# Autodesk Inventor assembly: ENSAMBLE_2
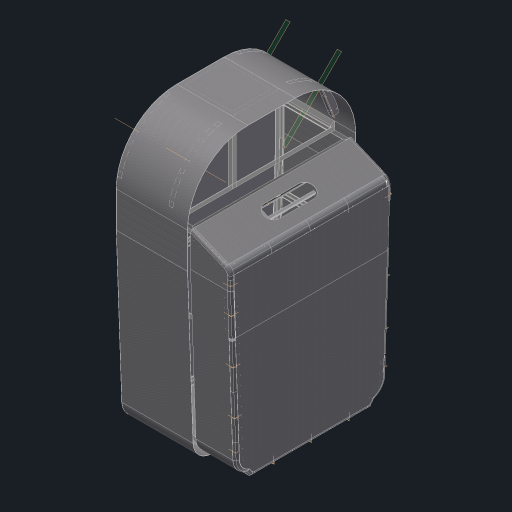
[picture p0: Inventor's stored thumbnail of the model, 512x512]
Saved by Autodesk Inventor 2024.3 (Build 283343000, 343)
## iProperties
Created: 2024-06-14
Part Number: ENSAMBLE_2
Material: Generic
Document SubType Name: Assembly
Designer: Niler
Author: Niler
## Documents named in this file (21)
- C:\Users\Niler\OneDrive\Escritorio\RECICLADOR\RECICLADOR_MODELO_3D\VERSION_3_COMPLETA\ENSAMBLE_2.iam
- C:\Users\Niler\OneDrive\Escritorio\RECICLADOR\RECICLADOR_MODELO_3D\VERSION_3_COMPLETA\CARCASA_ESTRUCTURA_Y_CHAPAS_2.iam
- C:\Users\Niler\OneDrive\Escritorio\RECICLADOR\RECICLADOR_MODELO_3D\VERSION_3_COMPLETA\PIEZAS_CHAPAS_ALUMINIO\CARCASA_ALUM_1.ipt
- C:\Users\Niler\OneDrive\Escritorio\RECICLADOR\RECICLADOR_MODELO_3D\VERSION_3_COMPLETA\ESQUINAS\ESQUINA_REDONDEADA_R20_P10.ipt
- C:\Users\Niler\OneDrive\Escritorio\RECICLADOR\RECICLADOR_MODELO_3D\VERSION_3_COMPLETA\ESQUINAS\ESQUINA_REDONDEADA_R20_P11.ipt
- C:\Users\Niler\OneDrive\Escritorio\RECICLADOR\RECICLADOR_MODELO_3D\VERSION_3_COMPLETA\ESQUINAS\ESQUINA_REDONDEADA_R20_P12.ipt
- C:\Users\Niler\OneDrive\Escritorio\RECICLADOR\RECICLADOR_MODELO_3D\VERSION_3_COMPLETA\NUEVAS_CHAPAS_ALUMINIO\CHAPA_1.ipt
- C:\Users\Niler\OneDrive\Escritorio\RECICLADOR\RECICLADOR_MODELO_3D\VERSION_3_COMPLETA\NUEVAS_CHAPAS_ALUMINIO\CHAPA_2.ipt
- C:\Users\Niler\OneDrive\Escritorio\RECICLADOR\RECICLADOR_MODELO_3D\VERSION_3_COMPLETA\NUEVAS_CHAPAS_ALUMINIO\CHAPA_3.ipt
- C:\Users\Niler\OneDrive\Escritorio\RECICLADOR\RECICLADOR_MODELO_3D\VERSION_3_COMPLETA\ESQUINAS\ESQUINA_REDONDEADA_R20_P5.ipt
- C:\Users\Niler\OneDrive\Escritorio\RECICLADOR\RECICLADOR_MODELO_3D\VERSION_3_COMPLETA\ESQUINAS\ESQUINA_REDONDEADA_R20_P13.ipt
- C:\Users\Niler\OneDrive\Escritorio\RECICLADOR\RECICLADOR_MODELO_3D\MECANISMO DE COMPACTADO\ENSAMBLE MECANISMO DE INGRESO.iam
- C:\Users\Niler\OneDrive\Escritorio\RECICLADOR\RECICLADOR_MODELO_3D\VERSION_3_COMPLETA\CURVA_SUPERIOR_IMPR.ipt
- C:\Users\Niler\OneDrive\Escritorio\RECICLADOR\RECICLADOR_MODELO_3D\VERSION_3_COMPLETA\ESQUINAS\ESQUINA_REDONDEADA_TRASERA.ipt
- C:\Users\Niler\OneDrive\Escritorio\RECICLADOR\RECICLADOR_MODELO_3D\VERSION_3_COMPLETA\ESQUINAS\ESQUINA_REDONDEADA_TRASERA_MIR.ipt
- C:\Users\Niler\OneDrive\Escritorio\RECICLADOR\RECICLADOR_MODELO_3D\VERSION_3_COMPLETA\CURVA_SUPERIOR_IMPR_MIR.ipt
- C:\Users\Niler\OneDrive\Escritorio\RECICLADOR\RECICLADOR_MODELO_3D\VERSION_3_COMPLETA\NUEVAS_CHAPAS_ALUMINIO\CHAPA_4_v2.ipt
- C:\Users\Niler\OneDrive\Escritorio\RECICLADOR\RECICLADOR_MODELO_3D\VERSION_3_COMPLETA\NUEVAS_CHAPAS_ALUMINIO\CHAPA_4_v2_MIR.ipt
- C:\Users\Niler\OneDrive\Escritorio\RECICLADOR\RECICLADOR_MODELO_3D\VERSION_3_COMPLETA\NUEVAS_CHAPAS_ALUMINIO\CHAPA_5.ipt
- C:\Users\Niler\OneDrive\Escritorio\RECICLADOR\RECICLADOR_MODELO_3D\VERSION_3_COMPLETA\ESQUINAS\ESQUINA_REDONDEADA_R20_P12_MIR.ipt
- C:\Users\Niler\OneDrive\Escritorio\RECICLADOR\RECICLADOR_MODELO_3D\VERSION_3_COMPLETA\NUEVAS_CHAPAS_ALUMINIO\CHAPA_6.ipt
## Components (30 placed, 20 different names)
1. CARCASA_ESTRUCTURA_Y_CHAPAS_2:1 [sub-assembly] — Flush:1, Mate:2, Mate:3, Mate:6, Mate:13, Mate:14, Mate:15, Mate:17, Mate:21, Mate:22, Mate:23, Mate:30, Mate:31, Mate:32, Mate:33, Mate:34, Mate:35, Mate:38, Mate:39, Flush:12, Mate:40, Flush:16, Mate:45, Flush:17, Mate:46, Mate:50, Mate:51, Flush:18
2. CARCASA_ALUM_1:1 — Flush:1, Mate:40, Mate:41, Mate:53
3. ESQUINA_REDONDEADA_R20_P10:1 — Mate:2, Mate:4, Mate:5, Mate:6, Mate:9, Flush:2, Mate:16
4. ESQUINA_REDONDEADA_R20_P11:1 — Mate:3, Mate:4, Mate:5, Mate:36
5. ESQUINA_REDONDEADA_R20_P10:2 — Mate:9, Flush:2, Flush:5, Mate:12, Flush:11
6. ESQUINA_REDONDEADA_R20_P11:2 — Flush:11, Mate:36, Mate:37
7. ESQUINA_REDONDEADA_R20_P10:3 — Flush:5, Mate:12
8. ESQUINA_REDONDEADA_R20_P11:3 — Mate:37
9. ESQUINA_REDONDEADA_R20_P12:1 — Mate:13, Mate:14, Mate:15
10. CHAPA_1:1 — Mate:33, Mate:34, Mate:35
11. CHAPA_2:1 — Mate:18, Flush:6
12. CHAPA_3:1 — Mate:16, Mate:17, Mate:18, Flush:6
13. ESQUINA_REDONDEADA_R20_P5:1 — Mate:22, Mate:27
14. ESQUINA_REDONDEADA_R20_P5:2 — Mate:21, Mate:23, Mate:26, Flush:9
15. ESQUINA_REDONDEADA_R20_P5:3 — Mate:27
16. ESQUINA_REDONDEADA_R20_P5:4 — Mate:26, Flush:9
17. ESQUINA_REDONDEADA_R20_P13:1 — Mate:28, Flush:10, Mate:29, Mate:30
18. ESQUINA_REDONDEADA_R20_P13:2 — Mate:28, Flush:10, Mate:29, Mate:31, Mate:32
19. ENSAMBLE MECANISMO DE INGRESO:1 [sub-assembly] — Mate:38, Mate:39
20. CURVA_SUPERIOR_IMPR:1 — Flush:12, Mate:41, Mate:44, Mate:47
21. CURVA_SUPERIOR_IMPR:3 — Mate:44, Flush:16, Mate:47, Flush:19
22. ESQUINA_REDONDEADA_TRASERA:1 — Mate:45, Flush:17, Mate:46, Mate:52
23. ESQUINA_REDONDEADA_TRASERA_MIR:1
24. CURVA_SUPERIOR_IMPR_MIR:1 — Mate:48, Mate:49
25. CURVA_SUPERIOR_IMPR_MIR:2 — Mate:48, Mate:49
26. CHAPA_4_v2:1 — Mate:50, Mate:51
27. CHAPA_4_v2_MIR:1
28. CHAPA_5:1 — Mate:52, Flush:18, Mate:53
29. ESQUINA_REDONDEADA_R20_P12_MIR:1
30. CHAPA_6:1 — Flush:19
## Relationships (64: Mate 50, Flush 14)
- Flush:1: CARCASA_ESTRUCTURA_Y_CHAPAS_2:1 ↔ CARCASA_ALUM_1:1
- Mate:2: CARCASA_ESTRUCTURA_Y_CHAPAS_2:1 ↔ ESQUINA_REDONDEADA_R20_P10:1
- Mate:3: CARCASA_ESTRUCTURA_Y_CHAPAS_2:1 ↔ ESQUINA_REDONDEADA_R20_P11:1
- Mate:4: ESQUINA_REDONDEADA_R20_P10:1 ↔ ESQUINA_REDONDEADA_R20_P11:1
- Mate:5: ESQUINA_REDONDEADA_R20_P10:1 ↔ ESQUINA_REDONDEADA_R20_P11:1
- Mate:6: CARCASA_ESTRUCTURA_Y_CHAPAS_2:1 ↔ ESQUINA_REDONDEADA_R20_P10:1
- [Mate]: ESQUINA_REDONDEADA_R20_P10:2 ↔ ESQUINA_REDONDEADA_R20_P11:2
- [Mate]: ESQUINA_REDONDEADA_R20_P10:2 ↔ ESQUINA_REDONDEADA_R20_P11:2
- Mate:9: ESQUINA_REDONDEADA_R20_P10:1 ↔ ESQUINA_REDONDEADA_R20_P10:2
- Flush:2: ESQUINA_REDONDEADA_R20_P10:1 ↔ ESQUINA_REDONDEADA_R20_P10:2
- [Mate]: ESQUINA_REDONDEADA_R20_P10:3 ↔ ESQUINA_REDONDEADA_R20_P11:3
- [Mate]: ESQUINA_REDONDEADA_R20_P10:3 ↔ ESQUINA_REDONDEADA_R20_P11:3
- Flush:5: ESQUINA_REDONDEADA_R20_P10:2 ↔ ESQUINA_REDONDEADA_R20_P10:3
- Mate:12: ESQUINA_REDONDEADA_R20_P10:2 ↔ ESQUINA_REDONDEADA_R20_P10:3
- Mate:13: CARCASA_ESTRUCTURA_Y_CHAPAS_2:1 ↔ ESQUINA_REDONDEADA_R20_P12:1
- Mate:14: CARCASA_ESTRUCTURA_Y_CHAPAS_2:1 ↔ ESQUINA_REDONDEADA_R20_P12:1
- Mate:15: CARCASA_ESTRUCTURA_Y_CHAPAS_2:1 ↔ ESQUINA_REDONDEADA_R20_P12:1
- Mate:16: ESQUINA_REDONDEADA_R20_P10:1 ↔ CHAPA_3:1
- Mate:17: CARCASA_ESTRUCTURA_Y_CHAPAS_2:1 ↔ CHAPA_3:1
- Mate:18: CHAPA_2:1 ↔ CHAPA_3:1
- Flush:6: CHAPA_2:1 ↔ CHAPA_3:1
- [Mate]: ESQUINA_REDONDEADA_R20_P5:1 ↔ ESQUINA_REDONDEADA_R20_P5:2
- [Flush]: ESQUINA_REDONDEADA_R20_P5:1 ↔ ESQUINA_REDONDEADA_R20_P5:2
- [Mate]: ESQUINA_REDONDEADA_R20_P5:1 ↔ ESQUINA_REDONDEADA_R20_P5:2
- Mate:21: CARCASA_ESTRUCTURA_Y_CHAPAS_2:1 ↔ ESQUINA_REDONDEADA_R20_P5:2
- Mate:22: CARCASA_ESTRUCTURA_Y_CHAPAS_2:1 ↔ ESQUINA_REDONDEADA_R20_P5:1
- Mate:23: CARCASA_ESTRUCTURA_Y_CHAPAS_2:1 ↔ ESQUINA_REDONDEADA_R20_P5:2
- [Mate]: ESQUINA_REDONDEADA_R20_P5:3 ↔ ESQUINA_REDONDEADA_R20_P5:4
- [Flush]: ESQUINA_REDONDEADA_R20_P5:3 ↔ ESQUINA_REDONDEADA_R20_P5:4
- [Mate]: ESQUINA_REDONDEADA_R20_P5:3 ↔ ESQUINA_REDONDEADA_R20_P5:4
- Mate:26: ESQUINA_REDONDEADA_R20_P5:2 ↔ ESQUINA_REDONDEADA_R20_P5:4
- Mate:27: ESQUINA_REDONDEADA_R20_P5:1 ↔ ESQUINA_REDONDEADA_R20_P5:3
- Flush:9: ESQUINA_REDONDEADA_R20_P5:2 ↔ ESQUINA_REDONDEADA_R20_P5:4
- Mate:28: ESQUINA_REDONDEADA_R20_P13:1 ↔ ESQUINA_REDONDEADA_R20_P13:2
- Flush:10: ESQUINA_REDONDEADA_R20_P13:1 ↔ ESQUINA_REDONDEADA_R20_P13:2
- Mate:29: ESQUINA_REDONDEADA_R20_P13:1 ↔ ESQUINA_REDONDEADA_R20_P13:2
- Mate:30: CARCASA_ESTRUCTURA_Y_CHAPAS_2:1 ↔ ESQUINA_REDONDEADA_R20_P13:1
- Mate:31: CARCASA_ESTRUCTURA_Y_CHAPAS_2:1 ↔ ESQUINA_REDONDEADA_R20_P13:2
- Mate:32: CARCASA_ESTRUCTURA_Y_CHAPAS_2:1 ↔ ESQUINA_REDONDEADA_R20_P13:2
- Mate:33: CARCASA_ESTRUCTURA_Y_CHAPAS_2:1 ↔ CHAPA_1:1
- Mate:34: CARCASA_ESTRUCTURA_Y_CHAPAS_2:1 ↔ CHAPA_1:1
- Mate:35: CARCASA_ESTRUCTURA_Y_CHAPAS_2:1 ↔ CHAPA_1:1
- Flush:11: ESQUINA_REDONDEADA_R20_P10:2 ↔ ESQUINA_REDONDEADA_R20_P11:2
- Mate:36: ESQUINA_REDONDEADA_R20_P11:1 ↔ ESQUINA_REDONDEADA_R20_P11:2
- Mate:37: ESQUINA_REDONDEADA_R20_P11:2 ↔ ESQUINA_REDONDEADA_R20_P11:3
- Mate:38: CARCASA_ESTRUCTURA_Y_CHAPAS_2:1 ↔ ENSAMBLE MECANISMO DE INGRESO:1
- Mate:39 (5 mm): CARCASA_ESTRUCTURA_Y_CHAPAS_2:1 ↔ ENSAMBLE MECANISMO DE INGRESO:1
- Flush:12: CARCASA_ESTRUCTURA_Y_CHAPAS_2:1 ↔ CURVA_SUPERIOR_IMPR:1
- Mate:40: CARCASA_ESTRUCTURA_Y_CHAPAS_2:1 ↔ CARCASA_ALUM_1:1
- Mate:41: CARCASA_ALUM_1:1 ↔ CURVA_SUPERIOR_IMPR:1
- Mate:44: CURVA_SUPERIOR_IMPR:1 ↔ CURVA_SUPERIOR_IMPR:3
- Flush:16: CARCASA_ESTRUCTURA_Y_CHAPAS_2:1 ↔ CURVA_SUPERIOR_IMPR:3
- Mate:45: CARCASA_ESTRUCTURA_Y_CHAPAS_2:1 ↔ ESQUINA_REDONDEADA_TRASERA:1
- Flush:17: CARCASA_ESTRUCTURA_Y_CHAPAS_2:1 ↔ ESQUINA_REDONDEADA_TRASERA:1
- Mate:46: CARCASA_ESTRUCTURA_Y_CHAPAS_2:1 ↔ ESQUINA_REDONDEADA_TRASERA:1
- Mate:47: CURVA_SUPERIOR_IMPR:1 ↔ CURVA_SUPERIOR_IMPR:3
- Mate:48: CURVA_SUPERIOR_IMPR_MIR:1 ↔ CURVA_SUPERIOR_IMPR_MIR:2
- Mate:49: CURVA_SUPERIOR_IMPR_MIR:1 ↔ CURVA_SUPERIOR_IMPR_MIR:2
- Mate:50: CARCASA_ESTRUCTURA_Y_CHAPAS_2:1 ↔ CHAPA_4_v2:1
- Mate:51: CARCASA_ESTRUCTURA_Y_CHAPAS_2:1 ↔ CHAPA_4_v2:1
- Mate:52: ESQUINA_REDONDEADA_TRASERA:1 ↔ CHAPA_5:1
- Flush:18: CARCASA_ESTRUCTURA_Y_CHAPAS_2:1 ↔ CHAPA_5:1
- Mate:53: CARCASA_ALUM_1:1 ↔ CHAPA_5:1
- Flush:19: CURVA_SUPERIOR_IMPR:3 ↔ CHAPA_6:1
## Named parameters: d8_d4 = 0 mm, d9_d5 = 0 mm, d13_d4 = 0 mm, d14_d5 = 0 mm, d38_d186 = 0 mm, d39_d187 = 0 mm, d40_d188 = 0 mm
